# Autodesk Inventor assembly: Suporte Superior
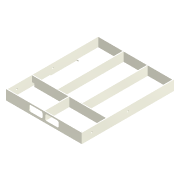
[picture p0: Inventor's stored thumbnail of the model, 180x180]
Saved by Autodesk Inventor 2020 (Build 240168000, 168)
## iProperties
Created: 2021-09-21
Part Number: Suporte Superior
Document SubType Name: Assembly
Designer: pablo
Author: pablo
## Documents named in this file (8)
- C:\Google Drive\Pablo Arquivos\Projetos\Utilidades Domesticas\Talheres\Suporte Superior.iam
- C:\Google Drive\Pablo Arquivos\Projetos\Utilidades Domesticas\Talheres\Divisória-22cm.ipt
- C:\Google Drive\Pablo Arquivos\Projetos\Utilidades Domesticas\Talheres\Divisória-25cm.ipt
- C:\Google Drive\Pablo Arquivos\Projetos\Utilidades Domesticas\Talheres\Divisória-24cm.ipt
- C:\Google Drive\Pablo Arquivos\Projetos\Utilidades Domesticas\Talheres\Divisória-7,5cm.ipt
- C:\Google Drive\Pablo Arquivos\Projetos\Utilidades Domesticas\Talheres\Divisória-25cm Frontal.ipt
- C:\Google Drive\Pablo Arquivos\Projetos\Utilidades Domesticas\Talheres\Divisória-30cm c rolamento - superior.ipt
- C:\Google Drive\Pablo Arquivos\Projetos\Utilidades Domesticas\Talheres\Base Superior.ipt
## Components (9 placed, 7 different names)
1. Divisória-22cm:1 — Mate:1, Mate:2
2. Divisória-22cm:2 — Mate:3, Mate:4
3. Divisória-25cm:2 — Mate:5, Mate:6
4. Divisória-24cm:1 — Mate:7, Mate:8, Mate:15, Mate:16
5. Divisória-7,5cm:1 — Mate:15, Mate:16, Mate:17
6. Divisória-25cm Frontal:1 — Mate:11, Mate:12
7. Divisória-30cm c rolamento - superior:1 — Mate:9, Mate:10
8. Base Superior:1 — Mate:1, Mate:2, Mate:3, Mate:4, Mate:5, Mate:6, Mate:7, Mate:8, Mate:9, Mate:10, Mate:11, Mate:12, Mate:13, Mate:14
9. Divisória-30cm c rolamento - superior:2 — Mate:13, Mate:14, Mate:17
## Relationships (17: Mate 17)
- Mate:1: Divisória-22cm:1 ↔ Base Superior:1
- Mate:2: Divisória-22cm:1 ↔ Base Superior:1
- Mate:3: Divisória-22cm:2 ↔ Base Superior:1
- Mate:4: Divisória-22cm:2 ↔ Base Superior:1
- Mate:5: Divisória-25cm:2 ↔ Base Superior:1
- Mate:6: Divisória-25cm:2 ↔ Base Superior:1
- Mate:7: Divisória-24cm:1 ↔ Base Superior:1
- Mate:8: Divisória-24cm:1 ↔ Base Superior:1
- Mate:9: Divisória-30cm c rolamento - superior:1 ↔ Base Superior:1
- Mate:10: Divisória-30cm c rolamento - superior:1 ↔ Base Superior:1
- Mate:11: Divisória-25cm Frontal:1 ↔ Base Superior:1
- Mate:12: Divisória-25cm Frontal:1 ↔ Base Superior:1
- Mate:13: Base Superior:1 ↔ Divisória-30cm c rolamento - superior:2
- Mate:14: Base Superior:1 ↔ Divisória-30cm c rolamento - superior:2
- Mate:15: Divisória-24cm:1 ↔ Divisória-7,5cm:1
- Mate:16: Divisória-24cm:1 ↔ Divisória-7,5cm:1
- Mate:17 (123.33 mm): Divisória-7,5cm:1 ↔ Divisória-30cm c rolamento - superior:2
